# Autodesk Inventor assembly: phalanx_plate
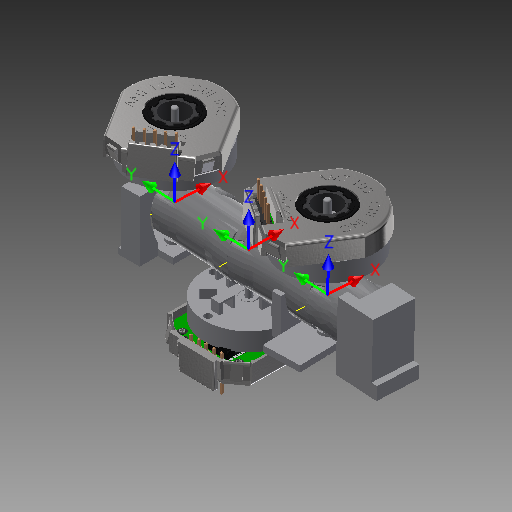
[picture p0: Inventor's stored thumbnail of the model, 512x512]
Saved by Autodesk Inventor 2019 (Build 230136000, 136)
## iProperties
Created: 2024-08-23
Part Number: phalanx_plate
Material: Generisch
Document SubType Name: Assembly
Designer: nic
Author: nic
## Documents named in this file (11)
- C:\Users\Nicolas Frick\Sync\OneDrive\wtm\nicol_rh8d\inventor\phalanx_plate.iam
- C:\Users\Nicolas Frick\Sync\OneDrive\wtm\nias\nias_description\inventor_files\hand\r_rh8d_refac\phalanx_refac.ipt
- C:\Users\Nicolas Frick\Sync\OneDrive\wtm\nicol_rh8d\inventor\phalanx_plate.ipt
- C:\Users\Nicolas Frick\Sync\OneDrive\wtm\nias\nias_description\inventor_files\hand\r_rh8d_refac\tip_refac.ipt
- C:\Users\Nicolas Frick\Sync\OneDrive\wtm\nicol_rh8d\inventor\tip_plate.ipt
- C:\Users\Nicolas Frick\Sync\OneDrive\wtm\nicol_rh8d\inventor\amt_socket_2mm.ipt
- C:\Users\Nicolas Frick\Sync\OneDrive\wtm\nicol_rh8d\inventor\Ballbearing.ipt
- C:\Users\Nicolas Frick\Sync\OneDrive\wtm\nicol_rh8d\inventor\shaft.ipt
- C:\Users\Nicolas Frick\Sync\OneDrive\wtm\nicol_rh8d\inventor\amt103-v unit only.ipt
- C:\Users\Nicolas Frick\Sync\OneDrive\wtm\nicol_rh8d\inventor\amt_plate.ipt
- C:\Users\Nicolas Frick\Sync\OneDrive\wtm\nicol_rh8d\inventor\finger_root_plate.ipt
## Components (22 placed, 10 different names)
1. phalanx_refac:1 — Fluchtend:2, Fluchtend:4, Passend:3, Passend:4, Passend:7, Fluchtend:5, Passend:8, Passend:9, Passend:23
2. phalanx_plate:1 — Fluchtend:2, Fluchtend:4, Passend:7, Fluchtend:5, Passend:21
3. phalanx_refac:2 — Passend:3, Passend:4, Passend:22, Passend:30
4. tip_refac:1 — Passend:8, Passend:9, Fluchtend:6, Fluchtend:7, Fluchtend:8
5. tip_plate:1 — Fluchtend:6, Fluchtend:7, Fluchtend:8
6. amt_socket_2mm:1 — Passend:10, Fluchtend:9, Fluchtend:10, Passend:20, Passend:29
7. amt_socket_2mm:2 — Passend:13, Fluchtend:12, Fluchtend:14, Passend:19, Passend:27
8. amt_socket_2mm:3 — Passend:12, Fluchtend:11, Fluchtend:13, Fluchtend:15, Passend:28
9. Ballbearing:1 — Passend:10, Fluchtend:9, Passend:11
10. shaft:1 — Passend:13, Passend:16, Passend:18, Passend:19, Passend:21, Passend:24
11. shaft:2 — Passend:12, Passend:15, Passend:17, Fluchtend:15, Passend:22, Passend:25, Fluchtend:16
12. shaft:3 — Passend:11, Passend:14, Passend:20, Passend:23, Passend:26, Passend:31, Passend:32
13. Ballbearing:2 — Passend:18, Fluchtend:14
14. Ballbearing:3 — Passend:17, Fluchtend:13
15. Ballbearing:4 — Passend:16, Fluchtend:12
16. Ballbearing:5 — Passend:15, Fluchtend:11
17. Ballbearing:6 — Passend:14, Fluchtend:10
18. amt103-v unit only:1 — Passend:24, Passend:27
19. amt103-v unit only:2 — Passend:25, Passend:28
20. amt103-v unit only:3 — Passend:26, Passend:29
21. amt_plate:1 — Passend:31, Passend:32
22. finger_root_plate:1 — Passend:30, Fluchtend:16
## Relationships (42: Mate 28, Flush 14)
- Fluchtend:2 [Flush]: phalanx_refac:1 ↔ phalanx_plate:1
- Fluchtend:4 [Flush] (-3.5 mm): phalanx_refac:1 ↔ phalanx_plate:1
- Passend:3 [Mate]: phalanx_refac:1 ↔ phalanx_refac:2
- Passend:4 [Mate] (0.8 mm): phalanx_refac:1 ↔ phalanx_refac:2
- Passend:7 [Mate]: phalanx_refac:1 ↔ phalanx_plate:1
- Fluchtend:5 [Flush] (3.5 mm): phalanx_refac:1 ↔ phalanx_plate:1
- Passend:8 [Mate]: phalanx_refac:1 ↔ tip_refac:1
- Passend:9 [Mate] (0.8 mm): phalanx_refac:1 ↔ tip_refac:1
- Fluchtend:6 [Flush]: tip_refac:1 ↔ tip_plate:1
- Fluchtend:7 [Flush]: tip_refac:1 ↔ tip_plate:1
- Fluchtend:8 [Flush]: tip_refac:1 ↔ tip_plate:1
- Passend:10 [Mate]: amt_socket_2mm:1 ↔ Ballbearing:1
- Fluchtend:9 [Flush]: amt_socket_2mm:1 ↔ Ballbearing:1
- Passend:11 [Mate]: Ballbearing:1 ↔ shaft:3
- Passend:12 [Mate]: amt_socket_2mm:3 ↔ shaft:2
- Passend:13 [Mate]: amt_socket_2mm:2 ↔ shaft:1
- Passend:14 [Mate]: shaft:3 ↔ Ballbearing:6
- Fluchtend:10 [Flush]: amt_socket_2mm:1 ↔ Ballbearing:6
- Passend:15 [Mate]: shaft:2 ↔ Ballbearing:5
- Fluchtend:11 [Flush]: amt_socket_2mm:3 ↔ Ballbearing:5
- Passend:16 [Mate]: shaft:1 ↔ Ballbearing:4
- Fluchtend:12 [Flush]: amt_socket_2mm:2 ↔ Ballbearing:4
- Passend:17 [Mate]: shaft:2 ↔ Ballbearing:3
- Fluchtend:13 [Flush]: amt_socket_2mm:3 ↔ Ballbearing:3
- Passend:18 [Mate]: shaft:1 ↔ Ballbearing:2
- Fluchtend:14 [Flush]: amt_socket_2mm:2 ↔ Ballbearing:2
- Passend:19 [Mate] (8 mm): amt_socket_2mm:2 ↔ shaft:1
- Passend:20 [Mate] (8 mm): amt_socket_2mm:1 ↔ shaft:3
- Fluchtend:15 [Flush] (-8 mm): amt_socket_2mm:3 ↔ shaft:2
- Passend:21 [Mate]: phalanx_plate:1 ↔ shaft:1
- Passend:22 [Mate]: phalanx_refac:2 ↔ shaft:2
- Passend:23 [Mate]: phalanx_refac:1 ↔ shaft:3
- Passend:24 [Mate]: shaft:1 ↔ amt103-v unit only:1
- Passend:25 [Mate]: shaft:2 ↔ amt103-v unit only:2
- Passend:26 [Mate]: shaft:3 ↔ amt103-v unit only:3
- Passend:27 [Mate]: amt_socket_2mm:2 ↔ amt103-v unit only:1
- Passend:28 [Mate]: amt_socket_2mm:3 ↔ amt103-v unit only:2
- Passend:29 [Mate]: amt_socket_2mm:1 ↔ amt103-v unit only:3
- Passend:30 [Mate]: phalanx_refac:2 ↔ finger_root_plate:1
- Passend:31 [Mate]: shaft:3 ↔ amt_plate:1
- Passend:32 [Mate]: shaft:3 ↔ amt_plate:1
- Fluchtend:16 [Flush]: shaft:2 ↔ finger_root_plate:1
